# Autodesk Inventor assembly: Connecting_Plate
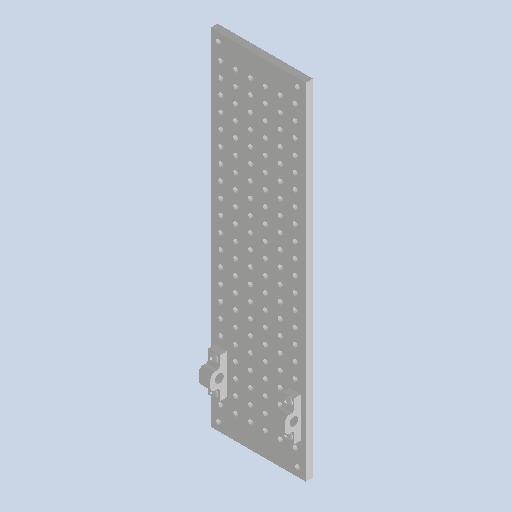
[picture p0: Inventor's stored thumbnail of the model, 512x512]
Saved by Autodesk Inventor 2024.1 (Build 281209000, 209)
## iProperties
Created: 2021-12-19
Part Number: Connecting_Plate
Document SubType Name: Assembly
Designer: muham
Author: muham
## Documents named in this file (5)
- C:\Users\udayk\OneDrive\Desktop\Year 1\Engineer IP13\Project 3\Thurs-08 Modelling\2. Hopper Assembly\2. Hopper Assembly\Connecting_Plate.iam
- C:\Users\udayk\OneDrive\Desktop\Year 1\Engineer IP13\Project 3\Thurs-08 Modelling\2. Hopper Assembly\2. Hopper Assembly\HopperVR41Y_Base.ipt
- C:\Users\udayk\OneDrive\Desktop\Year 1\Engineer IP13\Project 3\Thurs-08 Modelling\2. Hopper Assembly\2. Hopper Assembly\M4 x 16mm Machine Screw.ipt
- C:\Users\udayk\OneDrive\Desktop\Year 1\Engineer IP13\Project 3\Thurs-08 Modelling\2. Hopper Assembly\2. Hopper Assembly\M4 Nut.ipt
- C:\Users\udayk\OneDrive\Desktop\Year 1\Engineer IP13\Project 3\Thurs-08 Modelling\2. Hopper Assembly\2. Hopper Assembly\Modular_Single_Axle_V41Y.ipt
## Components (11 placed, 4 different names)
1. HopperVR41Y_Base:1 — Mate:17, Mate:18, Mate:19, Mate:20, Mate:21, Mate:22, Insert:9, Insert:10, Insert:11, Insert:12
2. Modular_Single_Axle_V41Y:1 — Mate:17, Mate:18, Mate:19, Insert:7, Insert:8
3. Modular_Single_Axle_V41Y:2 — Mate:20, Mate:21, Mate:22, Insert:5, Insert:6
4. M4 x 16mm Machine Screw:5 — Insert:5
5. M4 x 16mm Machine Screw:6 — Insert:6
6. M4 x 16mm Machine Screw:7 — Insert:7
7. M4 x 16mm Machine Screw:8 — Insert:8
8. M4 Nut:5 — Insert:9
9. M4 Nut:6 — Insert:10
10. M4 Nut:7 — Insert:11
11. M4 Nut:8 — Insert:12
## Relationships (14: Insert 8, Mate 6)
- Mate:17: HopperVR41Y_Base:1 ↔ Modular_Single_Axle_V41Y:1
- Mate:18: HopperVR41Y_Base:1 ↔ Modular_Single_Axle_V41Y:1
- Mate:19: HopperVR41Y_Base:1 ↔ Modular_Single_Axle_V41Y:1
- Mate:20: HopperVR41Y_Base:1 ↔ Modular_Single_Axle_V41Y:2
- Mate:21: HopperVR41Y_Base:1 ↔ Modular_Single_Axle_V41Y:2
- Mate:22: HopperVR41Y_Base:1 ↔ Modular_Single_Axle_V41Y:2
- Insert:5: Modular_Single_Axle_V41Y:2 ↔ M4 x 16mm Machine Screw:5
- Insert:6: Modular_Single_Axle_V41Y:2 ↔ M4 x 16mm Machine Screw:6
- Insert:7: Modular_Single_Axle_V41Y:1 ↔ M4 x 16mm Machine Screw:7
- Insert:8: Modular_Single_Axle_V41Y:1 ↔ M4 x 16mm Machine Screw:8
- Insert:9: HopperVR41Y_Base:1 ↔ M4 Nut:5
- Insert:10: HopperVR41Y_Base:1 ↔ M4 Nut:6
- Insert:11: HopperVR41Y_Base:1 ↔ M4 Nut:7
- Insert:12: HopperVR41Y_Base:1 ↔ M4 Nut:8
